# Autodesk Inventor assembly: bushing_assembly
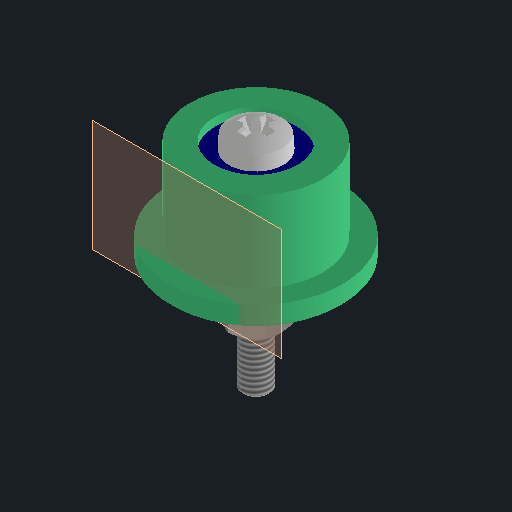
[picture p0: Inventor's stored thumbnail of the model, 512x512]
Saved by Autodesk Inventor 2024 (Build 280153000, 153)
## iProperties
Created: 2023-05-13
Part Number: bushing_assembly
Document SubType Name: Assembly
Designer: user
Author: user
## Documents named in this file (6)
- D:\Docs\Robot\3d\motor_assembly\bushing_assembly.iam
- D:\Docs\Robot\3d\motor_assembly\bushing_assembly\bushing.ipt
- D:\Docs\Robot\3d\default_components\604zz_bearing.ipt
- C:\Users\user\Documents\Inventor\Content Center Files\R2024\ru-RU\DIN 985\DIN 985 - M4.ipt
- C:\Users\user\Documents\Inventor\Content Center Files\R2024\ru-RU\DIN 7985 (H)\DIN 7985 (H) - M4x30-H.ipt
- C:\Users\user\Documents\Inventor\Content Center Files\R2024\ru-RU\DIN 934\DIN 934 - M4 x 0,7.ipt
## Components (5 placed, 5 different names)
1. bushing:1 — Совмещение:1, Совмещение:2, Совмещение:3, Вставка:1, Вставка:4
2. DIN 7985 (H) M4x30-H:1 — Вставка:2
3. 604zz_bearing:1 — Вставка:1, Вставка:2, Вставка:3
4. DIN 985 - заменено на DIN EN ISO 10511 M4:1 — Вставка:3
5. DIN 934 - заменено на DIN EN 24032/28673/28674 M4:1 — Вставка:4
## Relationships (7: Insert 4, Mate 3)
- Совмещение:1 [Mate]: bushing:1
- Совмещение:2 [Mate]: bushing:1
- Совмещение:3 [Mate]: bushing:1
- Вставка:1 [Insert]: bushing:1 ↔ 604zz_bearing:1
- Вставка:2 [Insert]: DIN 7985 (H) M4x30-H:1 ↔ 604zz_bearing:1
- Вставка:3 [Insert]: 604zz_bearing:1 ↔ DIN 985 - заменено на DIN EN ISO 10511 M4:1
- Вставка:4 [Insert] (7.8 mm): bushing:1 ↔ DIN 934 - заменено на DIN EN 24032/28673/28674 M4:1
